# Autodesk Inventor assembly: filament drive
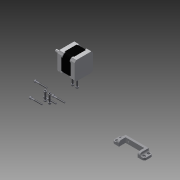
[picture p0: Inventor's stored thumbnail of the model, 180x180]
Saved by Autodesk Inventor 2013 (Build 170138000, 138)
## iProperties
Created: 2013-10-16
Part Number: filament drive
Document SubType Name: Assembly
Designer: employee
Author: employee
## Documents named in this file (14)
- C:\Users\employee\Desktop\ConceptFORGE\ConceptFORGE\Wally\INVENTOR\filament drive.iam
- C:\Users\employee\Desktop\ConceptFORGE\ConceptFORGE\Wally\INVENTOR\M3x25.ipt
- C:\Users\employee\Desktop\ConceptFORGE\ConceptFORGE\Wally\INVENTOR\stepper.ipt
- C:\Users\employee\Desktop\ConceptFORGE\ConceptFORGE\Wally\INVENTOR\m3 nut.ipt
- C:\Users\employee\Desktop\ConceptFORGE\ConceptFORGE\Wally\INVENTOR\M3x20.ipt
- C:\Users\employee\Desktop\ConceptFORGE\ConceptFORGE\FILAMENT DRIVE\INVENTOR FILES\BLOCK MIRROR.ipt
- C:\Users\employee\Desktop\ConceptFORGE\ConceptFORGE\FILAMENT DRIVE\INVENTOR FILES\WALLY MOUNT.ipt
- C:\Users\employee\Desktop\ConceptFORGE\ConceptFORGE\FILAMENT DRIVE\INVENTOR FILES\ARM MIRROR.ipt
- C:\Users\employee\Desktop\ConceptFORGE\ConceptFORGE\FILAMENT DRIVE\INVENTOR FILES\HOBBED PULLEY.ipt
- C:\Users\employee\Desktop\ConceptFORGE\ConceptFORGE\FILAMENT DRIVE\INVENTOR FILES\BEARING INSERT.ipt
- C:\Users\employee\Desktop\ConceptFORGE\ConceptFORGE\FILAMENT DRIVE\INVENTOR FILES\_608.ipt
- C:\Users\employee\Desktop\ConceptFORGE\ConceptFORGE\FILAMENT DRIVE\INVENTOR FILES\SPRING.ipt
- C:\Users\employee\Desktop\ConceptFORGE\ConceptFORGE\Wally\INVENTOR\M3x35.ipt
- C:\Users\employee\Desktop\ConceptFORGE\ConceptFORGE\Wally\INVENTOR\M3x30.ipt
## Components (27 placed, 13 different names)
1. M3x25:3 — Insert:13
2. M3x25:4 — Insert:14
3. stepper:1 — Insert:1, Angle:1, Insert:3, Mate:1, Flush:1, Angle:3
4. Hex Nut Metric M3 x 0.5:1 — Insert:11
5. Hex Nut Metric M3 x 0.5:2 — Insert:12
6. Hex Nut Metric M3 x 0.5:3 — Insert:9
7. Hex Nut Metric M3 x 0.5:4 — Insert:10
8. Forged Socket Head Cap Screw - Metric M3x0.5 x 20:1 — Insert:5
9. Forged Socket Head Cap Screw - Metric M3x0.5 x 20:2 — Insert:4
10. Forged Socket Head Cap Screw - Metric M3x0.5 x 20:3 — Insert:6
11. Forged Socket Head Cap Screw - Metric M3x0.5 x 20:4 — Insert:7
12. BLOCK MIRROR:1 — Insert:1, Angle:1, Insert:2, Insert:8, Insert:13, Insert:14, Insert:19, Insert:20
13. WALLY MOUNT:1 — Insert:2, Insert:4, Insert:5, Insert:6, Insert:7, Insert:8, Insert:9, Insert:10, Insert:11, Insert:12, Insert:22, Insert:23
14. ARM MIRROR:1 — Insert:3, Insert:16, Insert:17, Insert:18, Angle:2, Angle:3, Flush:2, Flush:3
15. HOBBED PULLEY:1 — Mate:1, Flush:1
16. BEARING INSERT:1 — Insert:15, Insert:16
17. _608:1 — Insert:15
18. SPRING:1 — Mate:3, Flush:2
19. SPRING:2 — Mate:2, Flush:3
20. M3x35:1 — Insert:19, Mate:3, Insert:21
21. M3x35:2 — Insert:20, Mate:2, Mate:4, Flush:4
22. Hex Nut Metric M3 x 0.5:5 — Insert:18, Angle:2
23. Hex Nut Metric M3 x 0.5:6 — Insert:21
24. Hex Nut Metric M3 x 0.5:7 — Mate:4, Flush:4
25. Forged Socket Head Cap Screw - Metric M3x0.5 x 20:5 — Insert:17
26. M3x30:1 — Insert:22
27. M3x30:2 — Insert:23
## Relationships (34: Insert 23, Mate 4, Flush 4, Angle 3)
- Insert:1: stepper:1 ↔ BLOCK MIRROR:1
- Angle:1 (0 deg): stepper:1 ↔ BLOCK MIRROR:1
- Insert:2: BLOCK MIRROR:1 ↔ WALLY MOUNT:1
- Insert:3: stepper:1 ↔ ARM MIRROR:1
- Insert:4 (12.5 mm): Forged Socket Head Cap Screw - Metric M3x0.5 x 20:2 ↔ WALLY MOUNT:1
- Insert:5 (12.5 mm): Forged Socket Head Cap Screw - Metric M3x0.5 x 20:1 ↔ WALLY MOUNT:1
- Insert:6 (12.5 mm): Forged Socket Head Cap Screw - Metric M3x0.5 x 20:3 ↔ WALLY MOUNT:1
- Insert:7 (12.5 mm): Forged Socket Head Cap Screw - Metric M3x0.5 x 20:4 ↔ WALLY MOUNT:1
- Insert:8: BLOCK MIRROR:1 ↔ WALLY MOUNT:1
- Insert:9: Hex Nut Metric M3 x 0.5:3 ↔ WALLY MOUNT:1
- Insert:10: Hex Nut Metric M3 x 0.5:4 ↔ WALLY MOUNT:1
- Insert:11: Hex Nut Metric M3 x 0.5:1 ↔ WALLY MOUNT:1
- Insert:12: Hex Nut Metric M3 x 0.5:2 ↔ WALLY MOUNT:1
- Insert:13: M3x25:3 ↔ BLOCK MIRROR:1
- Insert:14: M3x25:4 ↔ BLOCK MIRROR:1
- Mate:1: stepper:1 ↔ HOBBED PULLEY:1
- Flush:1 (-5.4 mm): stepper:1 ↔ HOBBED PULLEY:1
- Insert:15: BEARING INSERT:1 ↔ _608:1
- Insert:16: ARM MIRROR:1 ↔ BEARING INSERT:1
- Insert:17: ARM MIRROR:1 ↔ Forged Socket Head Cap Screw - Metric M3x0.5 x 20:5
- Insert:18: ARM MIRROR:1 ↔ Hex Nut Metric M3 x 0.5:5
- Angle:2 (0 deg): ARM MIRROR:1 ↔ Hex Nut Metric M3 x 0.5:5
- Insert:19: BLOCK MIRROR:1 ↔ M3x35:1
- Insert:20: BLOCK MIRROR:1 ↔ M3x35:2
- Angle:3 (0 deg): stepper:1 ↔ ARM MIRROR:1
- Mate:2: SPRING:2 ↔ M3x35:2
- Mate:3: SPRING:1 ↔ M3x35:1
- Flush:2: ARM MIRROR:1 ↔ SPRING:1
- Flush:3: ARM MIRROR:1 ↔ SPRING:2
- Mate:4: M3x35:2 ↔ Hex Nut Metric M3 x 0.5:7
- Insert:21 (-1.5 mm): M3x35:1 ↔ Hex Nut Metric M3 x 0.5:6
- Flush:4 (1.5 mm): M3x35:2 ↔ Hex Nut Metric M3 x 0.5:7
- Insert:22: WALLY MOUNT:1 ↔ M3x30:1
- Insert:23: WALLY MOUNT:1 ↔ M3x30:2
